# Autodesk Inventor assembly: mikrosumo
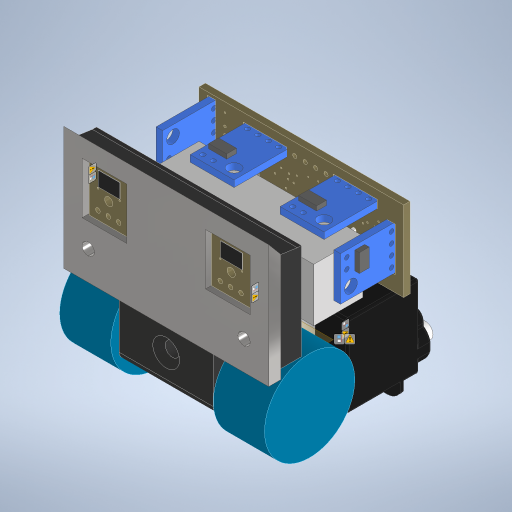
[picture p0: Inventor's stored thumbnail of the model, 512x512]
Saved by Autodesk Inventor 2023 (Build 270158000, 158)
## iProperties
Created: 2022-12-13
Part Number: mikrosumo
Document SubType Name: Assembly
Designer: komputer
Author: komputer
## Documents named in this file (11)
- C:\Users\Kamil\Desktop\MojeRoboty\BEETLE\beetle_mechanics\mikrosumo.iam
- C:\Users\Kamil\Desktop\MojeRoboty\BEETLE\beetle_mechanics\podsta.ipt
- C:\Users\Kamil\Desktop\MojeRoboty\BEETLE\beetle_mechanics\koło.ipt
- C:\Users\Kamil\Desktop\MojeRoboty\BEETLE\beetle_mechanics\opona.ipt
- C:\Users\Kamil\Desktop\MojeRoboty\BEETLE\beetle_mechanics\pokrywa silników.ipt
- C:\Users\Kamil\Desktop\MojeRoboty\BEETLE\beetle_mechanics\lipol 150mAH.ipt
- C:\Users\Kamil\Desktop\MojeRoboty\BEETLE\beetle_mechanics\nozz.ipt
- C:\Users\Kamil\Documents\Inventor\Miras_mechanics\servo_mini_1370hd_cos.ipt
- C:\Users\Kamil\Desktop\TOF_VLCOS.ipt
- C:\Users\Kamil\Desktop\MojeRoboty\BEETLE\beetle_mechanics\MikroSumo v2.ipt
- C:\Users\Kamil\Desktop\MojeRoboty\BEETLE\beetle_mechanics\ktir_plytka.ipt
## Components (17 placed, 10 different names)
1. podsta:1 — Flush:1, Mate:1, Flush:2, Zestawiające:10, Zestawiające:11, Zestawiające:12, Zestawiające:13
2. koło:1
3. koło:2
4. opona:1
5. opona:2
6. lipol 150mAH:1
7. nozz:1 — Równoległe:10, Równoległe:11
8. pokrywa silników:2 — Flush:1, Mate:1, Flush:2, Mate:3, Zestawiające:5, Zestawiające:6, Zestawiające:14
9. servo_mini_1370hd_cos:1 — Mate:3, Flush:7, Zestawiające:7, Równoległe:8, Równoległe:9
10. servo_mini_1370hd_cos:2 — Flush:7, Zestawiające:8, Równoległe:8, Równoległe:9, Zestawiające:9
11. TOF_VLCOS:1
12. TOF_VLCOS:2
13. TOF_VLCOS:3
14. TOF_VLCOS:5
15. MikroSumo v2:1 — Zestawiające:5, Zestawiające:6, Zestawiające:7, Zestawiające:8, Zestawiające:9, Zestawiające:14
16. ktir_plytka:2 — Zestawiające:10, Zestawiające:13, Równoległe:10
17. ktir_plytka:3 — Zestawiające:11, Zestawiające:12, Równoległe:11
## Relationships (19: Mate 12, Flush 7)
- Flush:1: podsta:1 ↔ pokrywa silników:2
- Mate:1 (11.5 mm): podsta:1 ↔ pokrywa silników:2
- Flush:2: podsta:1 ↔ pokrywa silników:2
- Mate:3: pokrywa silników:2 ↔ servo_mini_1370hd_cos:1
- Flush:7: servo_mini_1370hd_cos:1 ↔ servo_mini_1370hd_cos:2
- Zestawiające:5 [Mate]: pokrywa silników:2 ↔ MikroSumo v2:1
- Zestawiające:6 [Mate]: pokrywa silników:2 ↔ MikroSumo v2:1
- Zestawiające:7 [Mate]: servo_mini_1370hd_cos:1 ↔ MikroSumo v2:1
- Zestawiające:8 [Mate]: servo_mini_1370hd_cos:2 ↔ MikroSumo v2:1
- Równoległe:8 [Flush]: servo_mini_1370hd_cos:1 ↔ servo_mini_1370hd_cos:2
- Równoległe:9 [Flush]: servo_mini_1370hd_cos:1 ↔ servo_mini_1370hd_cos:2
- Zestawiające:9 [Mate]: servo_mini_1370hd_cos:2 ↔ MikroSumo v2:1
- Zestawiające:10 [Mate] (0.5 mm): podsta:1 ↔ ktir_plytka:2
- Zestawiające:11 [Mate] (0.5 mm): podsta:1 ↔ ktir_plytka:3
- Zestawiające:12 [Mate]: podsta:1 ↔ ktir_plytka:3
- Zestawiające:13 [Mate]: podsta:1 ↔ ktir_plytka:2
- Równoległe:10 [Flush] (-5 mm): nozz:1 ↔ ktir_plytka:2
- Równoległe:11 [Flush] (-5 mm): nozz:1 ↔ ktir_plytka:3
- Zestawiające:14 [Mate]: pokrywa silników:2 ↔ MikroSumo v2:1
